# Autodesk Inventor assembly: arm
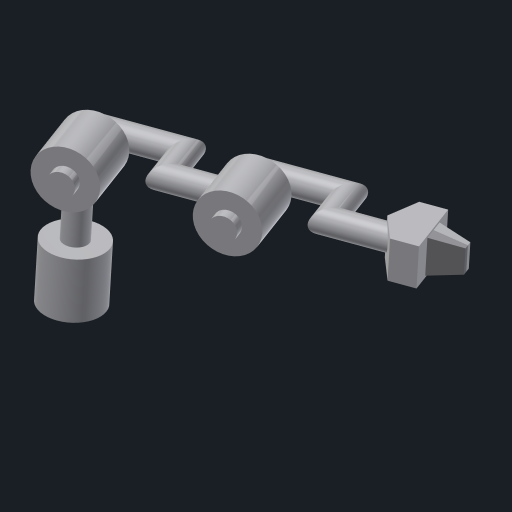
[picture p0: Inventor's stored thumbnail of the model, 512x512]
Saved by Autodesk Inventor 2023 (Build 270158000, 158)
## iProperties
Created: 2024-02-21
Part Number: arm
Document SubType Name: Assembly
Designer: valer
Author: valer
## Documents named in this file (7)
- C:\Users\valer\Desktop\basic_velocity_control\description\cad\arm.iam
- C:\Users\valer\Desktop\basic_velocity_control\description\cad\base.ipt
- C:\Users\valer\Desktop\basic_velocity_control\description\cad\upperarm.ipt
- C:\Users\valer\Desktop\basic_velocity_control\description\cad\forearm.ipt
- C:\Users\valer\Desktop\basic_velocity_control\description\cad\hand.ipt
- C:\Users\valer\Desktop\basic_velocity_control\description\cad\finger1.ipt
- C:\Users\valer\Desktop\basic_velocity_control\description\cad\finger2.ipt
## Components (6 placed, 6 different names)
1. base:1 — Flush:2, Mate:1, Mate:3, Mate:4
2. upperarm:1 — Mate:1, Mate:4, Flush:3, Angle:1
3. forearm:1 — Flush:3, Angle:2, Flush:4, Mate:5, Angle:3
4. hand:1 — Flush:4, Mate:5, Angle:3, Mate:6, Angle:4, Angle:5
5. finger1:1 — Mate:6, Angle:4, Angle:5
6. finger2:1
## Relationships (14: Mate 6, Angle 5, Flush 3)
- Flush:2: base:1
- Mate:1: base:1 ↔ upperarm:1
- [Mate]: upperarm:1 ↔ forearm:1
- Mate:3: base:1
- Mate:4: base:1 ↔ upperarm:1
- Flush:3: upperarm:1 ↔ forearm:1
- Angle:1 (0 deg): upperarm:1
- Angle:2 (0 deg): forearm:1
- Flush:4: forearm:1 ↔ hand:1
- Mate:5: forearm:1 ↔ hand:1
- Angle:3 (0 deg): forearm:1 ↔ hand:1
- Mate:6: hand:1 ↔ finger1:1
- Angle:4 (0 deg): hand:1 ↔ finger1:1
- Angle:5 (0 deg): hand:1 ↔ finger1:1
